# Autodesk Inventor assembly: v3.0
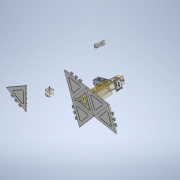
[picture p0: Inventor's stored thumbnail of the model, 180x180]
Saved by Autodesk Inventor 2022.3 (Build 263350000, 350)
## iProperties
Created: 2023-05-15
Part Number: v3.0
Document SubType Name: Assembly
Designer: Manuel Hueso Béjar
Author: Manuel Hueso Béjar
## Documents named in this file (15)
- C:\Users\Manuel Hueso Béjar\Desktop\3\2º Cuatrimestre\Robótica\2_Trabajo\CAD\v3.0\v3.0.iam
- C:\Users\Manuel Hueso Béjar\Desktop\3\2º Cuatrimestre\Robótica\2_Trabajo\CAD\v3.0\Base.ipt
- C:\Users\Manuel Hueso Béjar\Desktop\3\2º Cuatrimestre\Robótica\2_Trabajo\CAD\v3.0\Base2.ipt
- C:\Users\Manuel Hueso Béjar\Desktop\3\2º Cuatrimestre\Robótica\2_Trabajo\CAD\v3.0\Potenciómetro.ipt
- C:\Users\Manuel Hueso Béjar\Desktop\3\2º Cuatrimestre\Robótica\2_Trabajo\CAD\v3.0\Rod_1.ipt
- C:\Users\Manuel Hueso Béjar\Desktop\3\2º Cuatrimestre\Robótica\2_Trabajo\CAD\v3.0\Tube_1_1.ipt
- C:\Users\Manuel Hueso Béjar\Desktop\3\2º Cuatrimestre\Robótica\2_Trabajo\CAD\v3.0\Tube_1_2.ipt
- C:\Users\Manuel Hueso Béjar\Desktop\3\2º Cuatrimestre\Robótica\2_Trabajo\CAD\v3.0\Tube_2.ipt
- C:\Users\Manuel Hueso Béjar\Desktop\3\2º Cuatrimestre\Robótica\2_Trabajo\CAD\v3.0\Tube_3.ipt
- C:\Users\Manuel Hueso Béjar\Desktop\3\2º Cuatrimestre\Robótica\2_Trabajo\CAD\v3.0\Joint_Bearings.ipt
- C:\Users\Manuel Hueso Béjar\Downloads\rolling-bearing-lmxxuu-1.snapshot.6\roulement lmxxuu (ap203).ipt
- C:\Users\Manuel Hueso Béjar\Downloads\nema-17-motor-a-pasos-17hs4401-1-7amp-4kg-cm-1.snapshot.4\Nema 17 Motor a Pasos 17HS4401.iam
- C:\Users\Manuel Hueso Béjar\Downloads\timing-pulley-gt2-16-teeth-5mm-bore-2.snapshot.7\GT2-16T\GT2_16T.ipt
- C:\Users\Manuel Hueso Béjar\Desktop\3\2º Cuatrimestre\Robótica\2_Trabajo\CAD\v3.0\Joint_Tubes_1_2.ipt
- C:\Users\Manuel Hueso Béjar\Desktop\3\2º Cuatrimestre\Robótica\2_Trabajo\CAD\v3.0\Joint_Tubes_1_1.ipt
## Components (21 placed, 14 different names)
1. Base:1 — Rigid:1, Rigid:2, Rigid:3, Rotational:1, Rotational:2
2. Base2:1 — Rigid:1, Rigid:8
3. Base2:2 — Rigid:3
4. Base2:3 — Rigid:2
5. Base2:4
6. Base2:5 — Rigid:8
7. Potenciómetro:1 — Rotational:2
8. Rod_1:1 — Cylindrical:1, Rotational:7
9. Rod_1:2 — Cylindrical:2, Rotational:8
10. Tube_1_1:1 — Rotational:1, Rotational:3
11. Tube_1_2:1 — Rotational:3, Rigid:9, Rigid:10, Rigid:11
12. Tube_2:1 — Rotational:10
13. Tube_3:1 — Rotational:10
14. Joint_Bearings:1 — Rigid:6, Rigid:7
15. roulement lmxxuu (ap203):1 — Rigid:6, Cylindrical:1
16. roulement lmxxuu (ap203):2 — Rigid:7, Cylindrical:2
17. Nema 17 Motor a Pasos 17HS4401:1 [sub-assembly] — Rigid:9, Rotational:6
18. Nema 17 Motor a Pasos 17HS4401:2 [sub-assembly]
19. GT2_16T:1 — Rotational:6
20. Joint_Tubes_1_2:1 — Rigid:10, Rotational:7, Rotational:8
21. Joint_Tubes_1_1:1 — Rigid:11
## Relationships (18: WeldJoint 9, RevoluteJoint 7, CylindricalJoint 2)
- Rigid:1 [WeldJoint]: Base:1 ↔ Base2:1
- Rigid:2 [WeldJoint]: Base:1 ↔ Base2:3
- Rigid:3 [WeldJoint]: Base:1 ↔ Base2:2
- Rotational:1 [RevoluteJoint]: Base:1 ↔ Tube_1_1:1
- Rotational:2 [RevoluteJoint]: Base:1 ↔ Potenciómetro:1
- Rotational:3 [RevoluteJoint]: Tube_1_1:1 ↔ Tube_1_2:1
- Rigid:6 [WeldJoint] (1.5 mm): Joint_Bearings:1 ↔ roulement lmxxuu (ap203):1
- Rigid:7 [WeldJoint] (1.5 mm): Joint_Bearings:1 ↔ roulement lmxxuu (ap203):2
- Rigid:8 [WeldJoint]: Base2:1 ↔ Base2:5
- Cylindrical:1: Rod_1:1 ↔ roulement lmxxuu (ap203):1
- Cylindrical:2: Rod_1:2 ↔ roulement lmxxuu (ap203):2
- Rigid:9 [WeldJoint]: Tube_1_2:1 ↔ Nema 17 Motor a Pasos 17HS4401:1
- Rotational:6 [RevoluteJoint] (6 mm): Nema 17 Motor a Pasos 17HS4401:1 ↔ GT2_16T:1
- Rigid:10 [WeldJoint]: Tube_1_2:1 ↔ Joint_Tubes_1_2:1
- Rotational:7 [RevoluteJoint] (-3 mm): Rod_1:1 ↔ Joint_Tubes_1_2:1
- Rotational:8 [RevoluteJoint] (-3 mm): Rod_1:2 ↔ Joint_Tubes_1_2:1
- Rotational:10 [RevoluteJoint]: Tube_2:1 ↔ Tube_3:1
- Rigid:11 [WeldJoint]: Tube_1_2:1 ↔ Joint_Tubes_1_1:1
